# Autodesk Inventor assembly: test-model-2025stp3
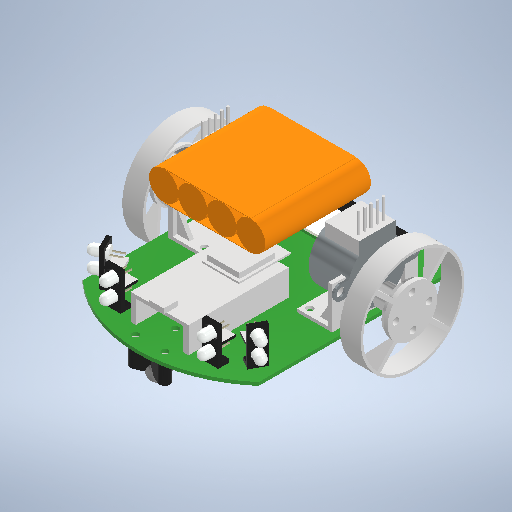
[picture p0: Inventor's stored thumbnail of the model, 512x512]
Saved by Autodesk Inventor 2025 (Build 290162000, 162)
## iProperties
Created: 2025-05-29
Part Number: test-model-2025stp3
Document SubType Name: Assembly
Designer: yamashita1
Author: yamashita1
## Documents named in this file (10)
- G:\マイドライブ\project\micro-mouse\3D-Model\test-model-2025stp3.iam
- G:\マイドライブ\project\micro-mouse\3D-Model\BallCaster-H16.ipt
- G:\マイドライブ\project\micro-mouse\3D-Model\Photo-Sensor.iam
- G:\マイドライブ\project\micro-mouse\3D-Model\ESP32-DevKitC.ipt
- G:\マイドライブ\project\micro-mouse\3D-Model\NiMH-Battery.ipt
- G:\マイドライブ\project\micro-mouse\3D-Model\AQM1602Y.ipt
- G:\マイドライブ\project\micro-mouse\3D-Model\Stepper-28BYJ_asm.iam
- G:\マイドライブ\project\micro-mouse\3D-Model\BaseBoard-stp3.ipt
- G:\マイドライブ\project\micro-mouse\3D-Model\Flange1.ipt
- G:\マイドライブ\project\micro-mouse\3D-Model\Wheel-D50A.ipt
## Components (16 placed, 9 different names)
1. BallCaster-H16:1 — メイト:7, メイト:8, メイト:9, 正接:1
2. Photo-Sensor:1 [sub-assembly] — メイト:15
3. Photo-Sensor:2 [sub-assembly] — メイト:14
4. Photo-Sensor:3 [sub-assembly] — メイト:12
5. Photo-Sensor:4 [sub-assembly] — メイト:13
6. ESP32-DevKitC:1 — メイト:10
7. NiMH-Battery:1
8. AQM1602Y:1 — メイト:11
9. Stepper-28BYJ_asm:1 [sub-assembly] — メイト:1, メイト:2, メイト:3, メイト:16, メイト:17
10. Stepper-28BYJ_asm:2 [sub-assembly] — メイト:4, メイト:5, メイト:6, メイト:18, メイト:19
11. BaseBoard-stp3:1 — メイト:1, メイト:2, メイト:3, メイト:4, メイト:5, メイト:6, メイト:7, メイト:8, メイト:9, メイト:10, 角度:1, メイト:11, メイト:12, メイト:13, メイト:14, メイト:15
12. BaseBoard-stp3:2 — 角度:1, 正接:1
13. Flange1:1 — メイト:16, メイト:17, メイト:20, メイト:21, メイト:22
14. Flange1:2 — メイト:18, メイト:19, メイト:23, メイト:24, メイト:25
15. Wheel-D50A:1 — メイト:20, メイト:21, メイト:22
16. Wheel-D50A:2 — メイト:23, メイト:24, メイト:25
## Relationships (27: Mate 25, Angle 1, Tangent 1)
- メイト:1 [Mate]: Stepper-28BYJ_asm:1 ↔ BaseBoard-stp3:1
- メイト:2 [Mate]: Stepper-28BYJ_asm:1 ↔ BaseBoard-stp3:1
- メイト:3 [Mate]: Stepper-28BYJ_asm:1 ↔ BaseBoard-stp3:1
- メイト:4 [Mate]: Stepper-28BYJ_asm:2 ↔ BaseBoard-stp3:1
- メイト:5 [Mate]: Stepper-28BYJ_asm:2 ↔ BaseBoard-stp3:1
- メイト:6 [Mate]: Stepper-28BYJ_asm:2 ↔ BaseBoard-stp3:1
- メイト:7 [Mate]: BallCaster-H16:1 ↔ BaseBoard-stp3:1
- メイト:8 [Mate]: BallCaster-H16:1 ↔ BaseBoard-stp3:1
- メイト:9 [Mate]: BallCaster-H16:1 ↔ BaseBoard-stp3:1
- メイト:10 [Mate]: ESP32-DevKitC:1 ↔ BaseBoard-stp3:1
- 角度:1 [Angle] (0 deg): BaseBoard-stp3:1 ↔ BaseBoard-stp3:2
- 正接:1 [Tangent]: BallCaster-H16:1 ↔ BaseBoard-stp3:2
- メイト:11 [Mate]: AQM1602Y:1 ↔ BaseBoard-stp3:1
- メイト:12 [Mate]: Photo-Sensor:3 ↔ BaseBoard-stp3:1
- メイト:13 [Mate]: Photo-Sensor:4 ↔ BaseBoard-stp3:1
- メイト:14 [Mate]: Photo-Sensor:2 ↔ BaseBoard-stp3:1
- メイト:15 [Mate]: Photo-Sensor:1 ↔ BaseBoard-stp3:1
- メイト:16 [Mate]: Stepper-28BYJ_asm:1 ↔ Flange1:1
- メイト:17 [Mate] (-7 mm): Stepper-28BYJ_asm:1 ↔ Flange1:1
- メイト:18 [Mate]: Stepper-28BYJ_asm:2 ↔ Flange1:2
- メイト:19 [Mate] (-7 mm): Stepper-28BYJ_asm:2 ↔ Flange1:2
- メイト:20 [Mate]: Flange1:1 ↔ Wheel-D50A:1
- メイト:21 [Mate]: Flange1:1 ↔ Wheel-D50A:1
- メイト:22 [Mate]: Flange1:1 ↔ Wheel-D50A:1
- メイト:23 [Mate]: Flange1:2 ↔ Wheel-D50A:2
- メイト:24 [Mate]: Flange1:2 ↔ Wheel-D50A:2
- メイト:25 [Mate]: Flange1:2 ↔ Wheel-D50A:2
